# Autodesk Inventor assembly: Robot Assembly
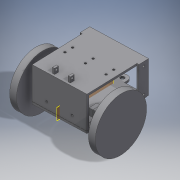
[picture p0: Inventor's stored thumbnail of the model, 180x180]
Saved by Autodesk Inventor 2018 (Build 220112000, 112)
## iProperties
Created: 2018-05-18
Part Number: Robot Assembly
Document SubType Name: Assembly
Designer: alexs
Author: alexs
## Documents named in this file (4)
- C:\Users\alexs\OneDrive\Documents\GitHub\ENGR101-AVC\Hardware CAD Files\Robot Assembly.iam
- C:\Users\alexs\OneDrive\Documents\GitHub\ENGR101-AVC\Hardware CAD Files\Wheel Base.ipt
- C:\Users\alexs\OneDrive\Documents\GitHub\ENGR101-AVC\Hardware CAD Files\Robot Base.ipt
- C:\Users\alexs\OneDrive\Documents\GitHub\ENGR101-AVC\Hardware CAD Files\Standard Parts\Wheel and Motor.ipt
## Components (4 placed, 3 different names)
1. Wheel Base:1 — Mate:1, Mate:2, Mate:3, Mate:4, Mate:5, Mate:6
2. Robot Base:1 — Mate:1, Mate:2
3. Wheel and Motor:1 — Mate:3, Mate:4
4. Wheel and Motor:2 — Mate:5, Mate:6
## Relationships (6: Mate 6)
- Mate:1: Wheel Base:1 ↔ Robot Base:1
- Mate:2: Wheel Base:1 ↔ Robot Base:1
- Mate:3: Wheel Base:1 ↔ Wheel and Motor:1
- Mate:4: Wheel Base:1 ↔ Wheel and Motor:1
- Mate:5: Wheel Base:1 ↔ Wheel and Motor:2
- Mate:6: Wheel Base:1 ↔ Wheel and Motor:2
